# Autodesk Inventor assembly: vl53l7cx-carrier-model
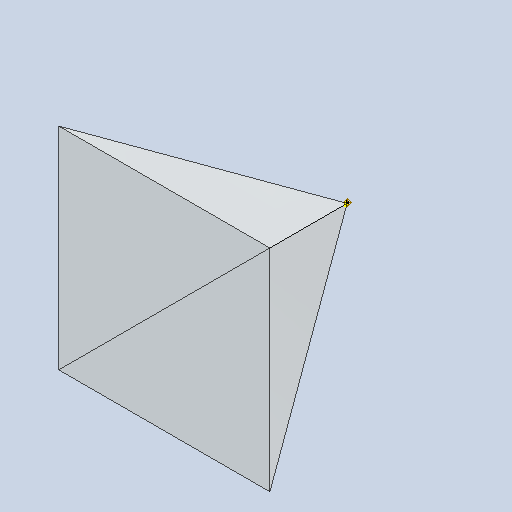
[picture p0: Inventor's stored thumbnail of the model, 512x512]
Saved by Autodesk Inventor 2025 (Build 290162000, 162)
## iProperties
Created: 2026-03-19
Part Number: vl53l7cx-carrier-model
Document SubType Name: Assembly
Designer: steve
Author: steve
## Documents named in this file (3)
- C:\Users\steve\Documents\Business\BunkScanner\Design\3D\vl53l7cx-carrier-model.iam
- C:\Users\steve\Documents\Business\BunkScanner\Design\3D\vl53l7cx-carrier-model.ipt
- C:\Users\steve\Documents\Business\BunkScanner\Design\3D\vl53l7cx-FOV.ipt
## Components (2 placed, 2 different names)
1. vl53l7cx-carrier-model:1 — Mate:1, Flush:1, Flush:2
2. vl53l7cx-FOV:1 — Mate:1, Flush:1, Flush:2
## Relationships (3: Flush 2, Mate 1)
- Mate:1: vl53l7cx-carrier-model:1 ↔ vl53l7cx-FOV:1
- Flush:1: vl53l7cx-carrier-model:1 ↔ vl53l7cx-FOV:1
- Flush:2: vl53l7cx-carrier-model:1 ↔ vl53l7cx-FOV:1
